# Autodesk Inventor assembly: SOPORTE LCD
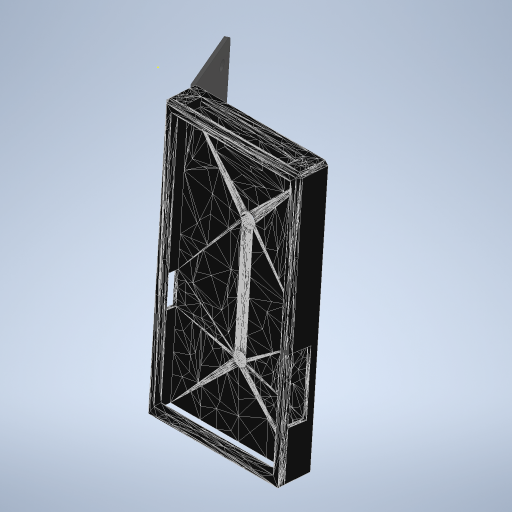
[picture p0: Inventor's stored thumbnail of the model, 512x512]
Saved by Autodesk Inventor 2023 (Build 270158000, 158)
## iProperties
Created: 2022-09-06
Part Number: SOPORTE LCD
Document SubType Name: Assembly
Designer: javie
Author: javie
## Documents named in this file (3)
- D:\Impresoras 3D\01-DOCUMENTOS TECNICOS\Modelo Ender 3\SOPORTE LCD.iam
- D:\Descargas\Imported Components\Main_Body_Phone_Holder_marked\Main_Body_Phone_Holder_marked.ipt
- D:\Impresoras 3D\01-DOCUMENTOS TECNICOS\Modelo Ender 3\LCD support_galaxy j5.ipt
## Components (2 placed, 2 different names)
1. Main_Body_Phone_Holder_marked:1 — Coincidencia:1, Coincidencia:2, Coincidencia:3
2. LCD support_galaxy j5:1 — Coincidencia:1, Coincidencia:2, Coincidencia:3
## Relationships (3: Mate 3)
- Coincidencia:1 [Mate]: Main_Body_Phone_Holder_marked:1 ↔ LCD support_galaxy j5:1
- Coincidencia:2 [Mate]: Main_Body_Phone_Holder_marked:1 ↔ LCD support_galaxy j5:1
- Coincidencia:3 [Mate]: Main_Body_Phone_Holder_marked:1 ↔ LCD support_galaxy j5:1
